# Autodesk Inventor assembly: 6060gantry
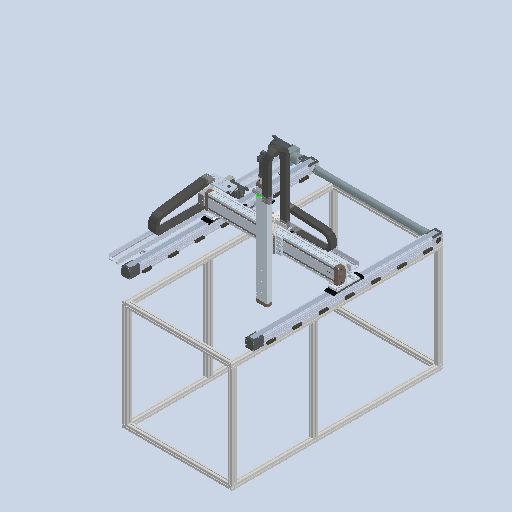
[picture p0: Inventor's stored thumbnail of the model, 512x512]
Saved by Autodesk Inventor 2022 (Build 260153000, 153)
## iProperties
Created: 2021-06-21
Part Number: 6060gantry
Document SubType Name: Assembly
Designer: lyndsaygreen
Author: lyndsaygreen
## Documents named in this file (4)
- \\Mac\Home\Desktop\WinnipegPMTTestFacility\gantry design\6060gantry.iam
- \\Mac\Home\Desktop\WinnipegPMTTestFacility\gantry design\GFS8-6060-1000_Autodesk_Inventor_2020_20210621\GFS8-6060-1000.ipt
- \\Mac\Home\Desktop\WinnipegPMTTestFacility\gantry design\GFS8-6060-1000_Autodesk_Inventor_2020_20210621\6060-5.5.ipt
- \\Mac\Home\Desktop\WinnipegPMTTestFacility\CMS_3SB_40_2_1820_1220_1020_10_10_20_MR.iam
## Components (15 placed, 3 different names)
1. GFS8-6060-1000:2 — Mate:1, Flush:1, Flush:2, Mate:3, Mate:6, Flush:11, Flush:12, Mate:7, Flush:13, Flush:14, Mate:14, Flush:24
2. GFS8-6060-1000:3 — Mate:17, Flush:29, Flush:30, Mate:18, Flush:31, Flush:32, Mate:20, Flush:34
3. GFS8-6060-1000:5 — Mate:2, Flush:3, Flush:4, Flush:5, Flush:6, Mate:4, Flush:7, Flush:8, Mate:5, Flush:9, Flush:10, Mate:13, Flush:23
4. GFS8-6060-1000:6 — Mate:15, Flush:25, Flush:26, Mate:16, Flush:27
5. 6060-5.5:1 — Mate:7, Flush:13, Flush:14, Flush:26, Mate:17, Flush:29, Flush:30
6. 6060-5.5:2 — Mate:13, Flush:23, Flush:33
7. 6060-5.5:3 — Mate:6, Flush:11, Flush:12, Mate:19
8. 6060-5.5:4 — Mate:14, Flush:24, Mate:19, Flush:33
9. 6060-5.5:5 — Mate:5, Flush:9, Flush:10, Flush:35
10. 6060-5.5:6 — Mate:4, Flush:7, Flush:8, Mate:15, Flush:25, Flush:28
11. 6060-5.5:7 — Mate:16, Flush:27, Flush:28
12. 6060-5.5:8 — Mate:3, Flush:5, Flush:6
13. 6060-5.5:9 — Mate:1, Flush:1, Flush:2, Mate:2, Flush:3, Flush:4
14. 6060-5.5:10 — Mate:18, Flush:31, Flush:32
15. CMS_3SB_40_2_1820_1220_1020_10_10_20_MR:1 [sub-assembly] — Mate:20, Flush:34, Flush:35
## Relationships (42: Flush 27, Mate 15)
- Mate:1: GFS8-6060-1000:2 ↔ 6060-5.5:9
- Flush:1: GFS8-6060-1000:2 ↔ 6060-5.5:9
- Flush:2: GFS8-6060-1000:2 ↔ 6060-5.5:9
- Mate:2: GFS8-6060-1000:5 ↔ 6060-5.5:9
- Flush:3: GFS8-6060-1000:5 ↔ 6060-5.5:9
- Flush:4: GFS8-6060-1000:5 ↔ 6060-5.5:9
- Mate:3: GFS8-6060-1000:2 ↔ 6060-5.5:8
- Flush:5: GFS8-6060-1000:5 ↔ 6060-5.5:8
- Flush:6: GFS8-6060-1000:5 ↔ 6060-5.5:8
- Mate:4: GFS8-6060-1000:5 ↔ 6060-5.5:6
- Flush:7: GFS8-6060-1000:5 ↔ 6060-5.5:6
- Flush:8: GFS8-6060-1000:5 ↔ 6060-5.5:6
- Mate:5: GFS8-6060-1000:5 ↔ 6060-5.5:5
- Flush:9: GFS8-6060-1000:5 ↔ 6060-5.5:5
- Flush:10: GFS8-6060-1000:5 ↔ 6060-5.5:5
- Mate:6: GFS8-6060-1000:2 ↔ 6060-5.5:3
- Flush:11: GFS8-6060-1000:2 ↔ 6060-5.5:3
- Flush:12: GFS8-6060-1000:2 ↔ 6060-5.5:3
- Mate:7: GFS8-6060-1000:2 ↔ 6060-5.5:1
- Flush:13: GFS8-6060-1000:2 ↔ 6060-5.5:1
- Flush:14: GFS8-6060-1000:2 ↔ 6060-5.5:1
- Mate:13: GFS8-6060-1000:5 ↔ 6060-5.5:2
- Flush:23: GFS8-6060-1000:5 ↔ 6060-5.5:2
- Mate:14: GFS8-6060-1000:2 ↔ 6060-5.5:4
- Flush:24: GFS8-6060-1000:2 ↔ 6060-5.5:4
- Mate:15: GFS8-6060-1000:6 ↔ 6060-5.5:6
- Flush:25: GFS8-6060-1000:6 ↔ 6060-5.5:6
- Flush:26: GFS8-6060-1000:6 ↔ 6060-5.5:1
- Mate:16: GFS8-6060-1000:6 ↔ 6060-5.5:7
- Flush:27: GFS8-6060-1000:6 ↔ 6060-5.5:7
- Flush:28: 6060-5.5:6 ↔ 6060-5.5:7
- Mate:17: GFS8-6060-1000:3 ↔ 6060-5.5:1
- Flush:29: GFS8-6060-1000:3 ↔ 6060-5.5:1
- Flush:30: GFS8-6060-1000:3 ↔ 6060-5.5:1
- Mate:18: GFS8-6060-1000:3 ↔ 6060-5.5:10
- Flush:31: GFS8-6060-1000:3 ↔ 6060-5.5:10
- Flush:32: GFS8-6060-1000:3 ↔ 6060-5.5:10
- Mate:19 (1524 mm): 6060-5.5:3 ↔ 6060-5.5:4
- Flush:33: 6060-5.5:2 ↔ 6060-5.5:4
- Mate:20: GFS8-6060-1000:3 ↔ CMS_3SB_40_2_1820_1220_1020_10_10_20_MR:1
- Flush:34: GFS8-6060-1000:3 ↔ CMS_3SB_40_2_1820_1220_1020_10_10_20_MR:1
- Flush:35: 6060-5.5:5 ↔ CMS_3SB_40_2_1820_1220_1020_10_10_20_MR:1
